# Autodesk Inventor assembly: High Strength Clamping Shaft Collar
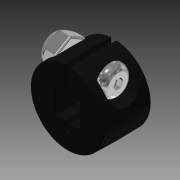
[picture p0: Inventor's stored thumbnail of the model, 180x180]
Saved by Autodesk Inventor 2016 SP2 (Build 200236200, 236)
## iProperties
Created: 2016-05-22
Part Number: High Strength Clamping Shaft Collar
Document SubType Name: Assembly
Designer: Jacob
Author: Jacob
## Documents named in this file (4)
- D:\Users\Owner\Desktop\Inventor Files\VEX Parts\Imperial\Motion\High Strength Clamping Shaft Collar.iam
- D:\Users\Owner\Desktop\Inventor Files\VEX Parts\Imperial\Motion\Components\276-3520-STEP.ipt
- D:\Users\Owner\Desktop\Inventor Files\VEX Parts\Imperial\Structure\Screw 8-32  x 0.625 inch long.ipt
- D:\Users\Owner\Desktop\Inventor Files\VEX Parts\Imperial\Structure\Nut 8-32 Nylock.ipt
## Components (3 placed, 3 different names)
1. 276-3520-STEP:1 — Insert:1, Mate:2
2. Hexagon Socket Button Head Cap Screw - Inch No. 8-36 - 5/8:1 — Insert:1, Mate:1
3. Nut 8-32 Nylock:1 — Mate:1, Mate:2
## Relationships (3: Mate 2, Insert 1)
- Insert:1: 276-3520-STEP:1 ↔ Hexagon Socket Button Head Cap Screw - Inch No. 8-36 - 5/8:1
- Mate:1: Hexagon Socket Button Head Cap Screw - Inch No. 8-36 - 5/8:1 ↔ Nut 8-32 Nylock:1
- Mate:2: 276-3520-STEP:1 ↔ Nut 8-32 Nylock:1
